# Autodesk Inventor assembly: Case_tray
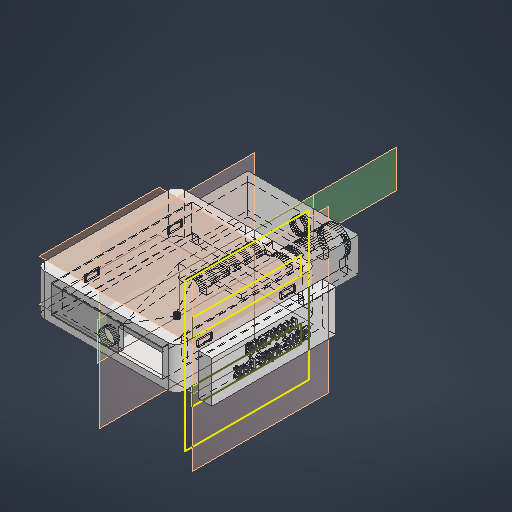
[picture p0: Inventor's stored thumbnail of the model, 512x512]
Saved by Autodesk Inventor 2026.1 (Build 301233020, 233B)
## iProperties
Created: 2025-11-04
Part Number: Case_tray
Document SubType Name: Assembly
Designer: sadi.canturk
Author: sadi.canturk
## Documents named in this file (3)
- C:\Users\sadi_\Documents\GitHub\Compact-NMR\System_development\magnet_design\B570_Tesla_magnet\CAD\Case_tray.iam
- C:\Users\sadi_\Documents\GitHub\Compact-NMR\System_development\magnet_design\B570_Tesla_magnet\CAD\BaseCase_AlignmentSupport.ipt
- C:\Users\sadi_\Documents\GitHub\Compact-NMR\System_development\magnet_design\B570_Tesla_magnet\CAD\tray.ipt
## Components (2 placed, 2 different names)
1. BaseCase_AlignmentSupport:1 — Flush:2, Mate:2, Mate:3
2. tray:1 — Flush:2, Mate:2, Mate:3
## Relationships (3: Mate 2, Flush 1)
- Flush:2: BaseCase_AlignmentSupport:1 ↔ tray:1
- Mate:2 (0.1 mm): BaseCase_AlignmentSupport:1 ↔ tray:1
- Mate:3 (0.3 mm): BaseCase_AlignmentSupport:1 ↔ tray:1
